# Autodesk Inventor assembly: outside6motorbearing
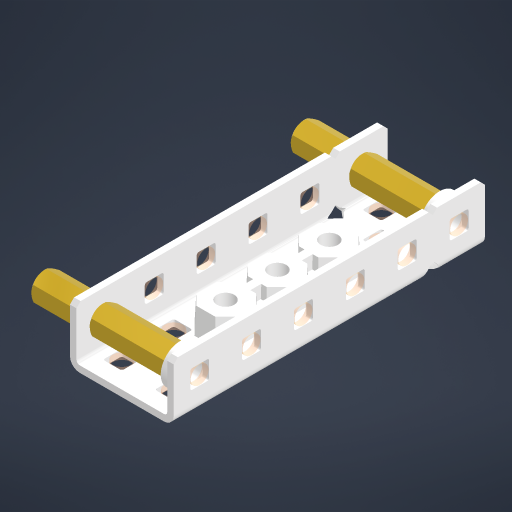
[picture p0: Inventor's stored thumbnail of the model, 512x512]
Saved by Autodesk Inventor 2023 (Build 270158000, 158)
## iProperties
Created: 2023-08-06
Part Number: outside6motorbearing
Document SubType Name: Assembly
Designer: srbel
Author: srbel
## Documents named in this file (8)
- C:\CAD\OverUnderCAD\Drive\outside6motorbearing.iam
- C:\CAD\OverUnderCAD\VEX-CAD-Inventor-1.4.0\Structure\C Channel\Aluminum 1x2x1\Alu C 1x2x1x6.ipt
- C:\CAD\OverUnderCAD\VEX-CAD-Inventor-1.4.0\Structure\Standoff\Standoff .50.ipt
- C:\CAD\OverUnderCAD\VEX-CAD-Inventor-1.4.0\Structure\Standoff.ipt
- C:\CAD\OverUnderCAD\VEX-CAD-Inventor-1.4.0\Structure\Standoff\Standoff .75.ipt
- C:\CAD\OverUnderCAD\VEX-CAD-Inventor-1.4.0\Motion\Spacers\Spacer Nylon .313 OD\NSpacer .313 OD x .125.ipt
- C:\CAD\OverUnderCAD\VEX-CAD-Inventor-1.4.0\Motion\Spacers\Spacer Nylon .313 OD.ipt
- C:\CAD\OverUnderCAD\VEX-CAD-Inventor-1.4.0\Motion\Shaft LS\Bearing Flat.ipt
## Components (8 placed, 5 different names)
1. Alu C 1x2x1x6:1 — Insert:1, Insert:2, Insert:3, Insert:4, Insert:7, Insert:8
2. Standoff .50:1 — Insert:1
3. Standoff .50:2 — Insert:2
4. Standoff .75:3 — Insert:3, Insert:5
5. Standoff .75:4 — Insert:4, Insert:6
6. NSpacer .313 OD x .125:1 — Insert:6
7. NSpacer .313 OD x .125:2 — Insert:5
8. Bearing Flat:1 — Insert:7, Insert:8
## Relationships (8: Insert 8)
- Insert:1: Alu C 1x2x1x6:1 ↔ Standoff .50:1
- Insert:2: Alu C 1x2x1x6:1 ↔ Standoff .50:2
- Insert:3: Alu C 1x2x1x6:1 ↔ Standoff .75:3
- Insert:4: Alu C 1x2x1x6:1 ↔ Standoff .75:4
- Insert:5: Standoff .75:3 ↔ NSpacer .313 OD x .125:2
- Insert:6: Standoff .75:4 ↔ NSpacer .313 OD x .125:1
- Insert:7: Alu C 1x2x1x6:1 ↔ Bearing Flat:1
- Insert:8: Alu C 1x2x1x6:1 ↔ Bearing Flat:1
